# Autodesk Inventor assembly: assm
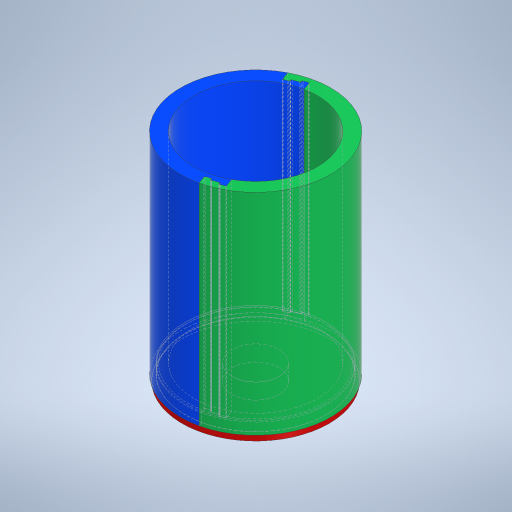
[picture p0: Inventor's stored thumbnail of the model, 512x512]
Saved by Autodesk Inventor 2024 (Build 280153000, 153)
## iProperties
Created: 2023-10-17
Part Number: assm
Document SubType Name: Assembly
Designer: Pokemba2
Author: Pokemba2
## Documents named in this file (4)
- C:\Users\Pokemba2\Desktop\NAKUJA\mould 4.0\assm.iam
- C:\Users\Pokemba2\Desktop\NAKUJA\mould 4.0\base.ipt
- C:\Users\Pokemba2\Desktop\NAKUJA\mould 4.0\cyl inner.ipt
- C:\Users\Pokemba2\Desktop\NAKUJA\mould 4.0\cyl outer.ipt
## Components (3 placed, 3 different names)
1. base:1 — Mate:3, Mate:4
2. cyl inner:1 — Flush:1, Mate:1, Mate:2
3. cyl outer:1 — Flush:1, Mate:1, Mate:2, Mate:3, Mate:4
## Relationships (5: Mate 4, Flush 1)
- Flush:1: cyl inner:1 ↔ cyl outer:1
- Mate:1: cyl inner:1 ↔ cyl outer:1
- Mate:2: cyl inner:1 ↔ cyl outer:1
- Mate:3: base:1 ↔ cyl outer:1
- Mate:4: base:1 ↔ cyl outer:1
